# Autodesk Inventor assembly: component box all
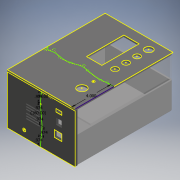
[picture p0: Inventor's stored thumbnail of the model, 180x180]
Saved by Autodesk Inventor 2021 (Build 250183000, 183)
## iProperties
Created: 2023-01-12
Part Number: component box all
Document SubType Name: Assembly
Designer: boyle
Author: boyle
## Documents named in this file (5)
- C:\Users\boyle\OneDrive\Documents\college\EExxx\EE420\SD boxes\component box all.iam
- C:\Users\boyle\OneDrive\Documents\college\EExxx\EE420\SD boxes\Component box Bottom.ipt
- C:\Users\boyle\OneDrive\Documents\college\EExxx\EE420\SD boxes\component box cover.ipt
- C:\Users\boyle\OneDrive\Documents\college\EExxx\EE420\SD boxes\Component box top.ipt
- C:\Users\boyle\OneDrive\Documents\college\EExxx\EE420\SD boxes\compnent box front.ipt
## Components (4 placed, 4 different names)
1. Component box Bottom:1 — Mate:1, Flush:1, Flush:2
2. Component box top:1 — Mate:1, Flush:1, Flush:2, Flush:3, Flush:4, Mate:2, Flush:6, Flush:7
3. component box cover:1 — Mate:2, Flush:5, Flush:6, Flush:7
4. compnent box front:1 — Flush:3, Flush:4, Flush:5
## Relationships (9: Flush 7, Mate 2)
- Mate:1: Component box Bottom:1 ↔ Component box top:1
- Flush:1: Component box Bottom:1 ↔ Component box top:1
- Flush:2: Component box Bottom:1 ↔ Component box top:1
- Flush:3: Component box top:1 ↔ compnent box front:1
- Flush:4: Component box top:1 ↔ compnent box front:1
- Mate:2: Component box top:1 ↔ component box cover:1
- Flush:5: component box cover:1 ↔ compnent box front:1
- Flush:6: Component box top:1 ↔ component box cover:1
- Flush:7: Component box top:1 ↔ component box cover:1
